# Autodesk Inventor assembly: UQ203-topHolder-sample
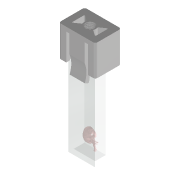
[picture p0: Inventor's stored thumbnail of the model, 180x180]
Saved by Autodesk Inventor 2021 (Build 250183000, 183)
## iProperties
Created: 2023-02-10
Part Number: UQ203-topHolder-sample
Document SubType Name: Assembly
Designer: nvladi
Author: nvladi
## Documents named in this file (4)
- C:\Users\Public\GitHub-public\benchtop-hardware\Benchtop\CAD-model-Inventor2021\mesoSPIM\sample_handling\assemblies\UQ203-topHolder-sample.iam
- C:\Users\Public\GitHub-public\benchtop-hardware\Benchtop\CAD-model-Inventor2021\mesoSPIM\sample_handling\cuvette-holders\Cuvette-7.5x12.5mm(UG203)\Clamp-UG203_100943(12.5 x 7.5mm)_E.ipt
- C:\Users\Public\GitHub-public\benchtop-hardware\Benchtop\CAD-model-Inventor2021\library\Portmann Instruments\UQ-203-5x10x45mm.ipt
- C:\Users\Public\GitHub-public\benchtop-hardware\Benchtop\CAD-model-Inventor2021\mesoSPIM\sample_handling\cuvette-clamps\Cuvette-7.5x12.5mm(UG203)\kidney-7mm.ipt
## Components (3 placed, 3 different names)
1. Clamp-UG203_100943(12.5 x 7.5mm)_E:1 — Mate:1, Flush:1, Flush:2
2. UQ-203-5x10x45mm:1 — Mate:1, Flush:1, Flush:2
3. kidney-7mm:1
## Relationships (3: Flush 2, Mate 1)
- Mate:1: Clamp-UG203_100943(12.5 x 7.5mm)_E:1 ↔ UQ-203-5x10x45mm:1
- Flush:1 (-2.25 mm): Clamp-UG203_100943(12.5 x 7.5mm)_E:1 ↔ UQ-203-5x10x45mm:1
- Flush:2 (-2.25 mm): Clamp-UG203_100943(12.5 x 7.5mm)_E:1 ↔ UQ-203-5x10x45mm:1
